# Autodesk Inventor assembly: DriveHousing
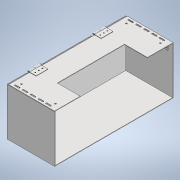
[picture p0: Inventor's stored thumbnail of the model, 180x180]
Saved by Autodesk Inventor 2020 (Build 240168000, 168)
## iProperties
Created: 2021-11-11
Part Number: DriveHousing
Document SubType Name: Assembly
Designer: 17185
Author: 17185
## Documents named in this file (6)
- C:\Users\17185\Desktop\chassis draft\DriveHousing.iam
- C:\Users\17185\Desktop\chassis draft\DriveHousing.ipt
- C:\Users\17185\Desktop\chassis draft\Hinge\leaf.ipt
- C:\Users\17185\Desktop\chassis draft\Hinge\Pin.ipt
- C:\Users\17185\Desktop\chassis draft\lid.ipt
- C:\Users\17185\Desktop\chassis draft\CornerBrace.ipt
## Components (12 placed, 5 different names)
1. DriveHousing:1 — Mate:1, Mate:2, Flush:5, Flush:6, Mate:28, Mate:30, Mate:33, Mate:34
2. leaf:1 — Mate:1, Mate:3, Flush:1, Flush:6
3. leaf:2 — Mate:2, Mate:4, Flush:2
4. Pin:1 — Mate:4, Flush:2, Flush:4, Mate:6
5. Pin:2 — Mate:3, Flush:1, Flush:3, Mate:5
6. leaf:3 — Flush:4, Mate:6, Flush:5, Mate:11, Mate:13
7. leaf:4 — Flush:3, Mate:5, Mate:12, Mate:14
8. lid:1 — Mate:11, Mate:12, Mate:13, Mate:14, Mate:29, Mate:31, Mate:32, Mate:35
9. CornerBrace:1 — Mate:34, Mate:35
10. CornerBrace:2 — Mate:32, Mate:33
11. CornerBrace:3 — Mate:28, Mate:29
12. CornerBrace:4 — Mate:30, Mate:31
## Relationships (24: Mate 18, Flush 6)
- Mate:1: DriveHousing:1 ↔ leaf:1
- Mate:2: DriveHousing:1 ↔ leaf:2
- Mate:3: leaf:1 ↔ Pin:2
- Mate:4: leaf:2 ↔ Pin:1
- Flush:1: leaf:1 ↔ Pin:2
- Flush:2: leaf:2 ↔ Pin:1
- Flush:3: Pin:2 ↔ leaf:4
- Flush:4: Pin:1 ↔ leaf:3
- Mate:5: Pin:2 ↔ leaf:4
- Mate:6: Pin:1 ↔ leaf:3
- Flush:5 (-134.112 mm): DriveHousing:1 ↔ leaf:3
- Flush:6 (-134.112 mm): DriveHousing:1 ↔ leaf:1
- Mate:11: leaf:3 ↔ lid:1
- Mate:12: leaf:4 ↔ lid:1
- Mate:13: leaf:3 ↔ lid:1
- Mate:14: leaf:4 ↔ lid:1
- Mate:28: DriveHousing:1 ↔ CornerBrace:3
- Mate:29: lid:1 ↔ CornerBrace:3
- Mate:30: DriveHousing:1 ↔ CornerBrace:4
- Mate:31: lid:1 ↔ CornerBrace:4
- Mate:32: lid:1 ↔ CornerBrace:2
- Mate:33: DriveHousing:1 ↔ CornerBrace:2
- Mate:34: DriveHousing:1 ↔ CornerBrace:1
- Mate:35: lid:1 ↔ CornerBrace:1
